# Autodesk Inventor assembly: mini predator camera block for boolian
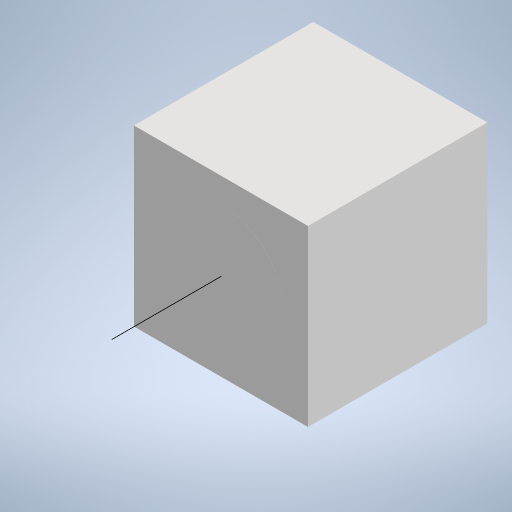
[picture p0: Inventor's stored thumbnail of the model, 512x512]
Saved by Autodesk Inventor 2023 (Build 270158000, 158)
## iProperties
Created: 2023-02-19
Part Number: mini predator camera block for boolian
Document SubType Name: Assembly
Designer: Steven
Author: Steven
## Documents named in this file (3)
- Y:\FPV drone stuff\0 Street League\Frames\PB-Kauri-X\3D prints\35 mm canopy\work in progress prints\Camera mounts\predator mini\mini predator camera block for boolian.iam
- Y:\FPV drone stuff\0 Street League\Frames\PB-Kauri-X\3D prints\35 mm canopy\work in progress prints\Camera mounts\predator mini\mini predator camera block.ipt
- Y:\FPV drone stuff\0 Street League\Frames\PB-Kauri-X\3D prints\35 mm canopy\work in progress prints\Camera mounts\predator mini\mini predator dummy camera.ipt
## Components (2 placed, 2 different names)
1. mini predator camera block:1 — Flush:1, Flush:2, Flush:3, Flush:4, Flush:5, Flush:6
2. mini predator dummy camera:1 — Flush:4, Flush:5, Flush:6
## Relationships (6: Flush 6)
- Flush:1: mini predator camera block:1
- Flush:2: mini predator camera block:1
- Flush:3: mini predator camera block:1
- Flush:4 (2 mm): mini predator camera block:1 ↔ mini predator dummy camera:1
- Flush:5 (2 mm): mini predator camera block:1 ↔ mini predator dummy camera:1
- Flush:6: mini predator camera block:1 ↔ mini predator dummy camera:1
